# Autodesk Inventor assembly: motor_assembly_S_MIR
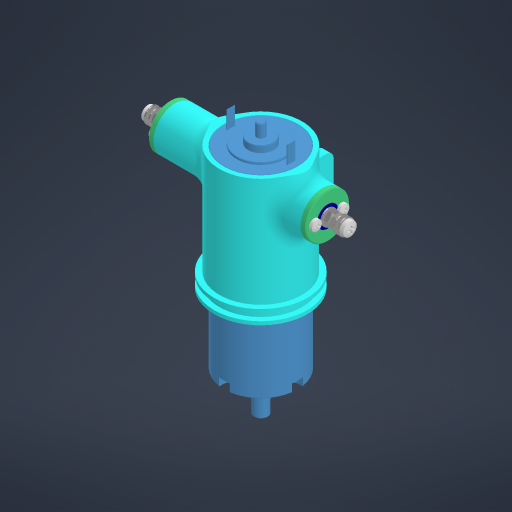
[picture p0: Inventor's stored thumbnail of the model, 512x512]
Saved by Autodesk Inventor 2024 (Build 280153000, 153)
## iProperties
Created: 2023-04-15
Part Number: motor_assembly_S_MIR
Document SubType Name: Assembly
Designer: user
Author: user
## Documents named in this file (4)
- D:\Docs\Robot\3d\motor_assembly\side\motor_assembly_S_MIR.iam
- D:\Docs\Robot\3d\default_components\motor_MIR.ipt
- D:\Docs\Robot\3d\motor_assembly\side\lower_arm_MIR.ipt
- D:\Docs\Robot\3d\motor_assembly\bushing_assembly\bushing_assembly.iam
## Components (4 placed, 3 different names)
1. motor_MIR:1 — Совмещение:3, Совмещение:2, Совмещение:1, Заподлицо:1
2. lower_arm_MIR:1 — Совмещение:4, Заподлицо:1, Вставка:1, Совмещение:6
3. bushing_assembly:1 [sub-assembly] — Совмещение:6
4. bushing_assembly:2 [sub-assembly] — Вставка:1
## Relationships (7: Mate 6, Insert 1)
- Совмещение:3 [Mate]: motor_MIR:1
- Совмещение:2 [Mate]: motor_MIR:1
- Совмещение:1 [Mate]: motor_MIR:1
- Совмещение:4 [Mate]: lower_arm_MIR:1
- Заподлицо:1 [Mate]: motor_MIR:1 ↔ lower_arm_MIR:1
- Вставка:1 [Insert]: lower_arm_MIR:1 ↔ bushing_assembly:2
- Совмещение:6 [Mate]: lower_arm_MIR:1 ↔ bushing_assembly:1
